# Autodesk Inventor assembly: ma2010_asm
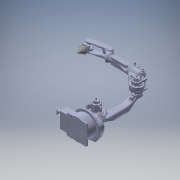
[picture p0: Inventor's stored thumbnail of the model, 180x180]
Saved by Autodesk Inventor 2017 (Build 210142000, 142)
## iProperties
Created: 2020-12-29
Part Number: ma2010_asm
Material: 一般
Document SubType Name: Assembly
Designer: Brian
Sending System: Autodesk Inventor 2020
Preprocessor: ST-DEVELOPER v18
Title: F:\DesktopSpace\MASTERS\ma2010_asm.stp
Author: Crowm
Revision Number: ANY
## Documents named in this file (9)
- E:\Brian\暫存\新增資料夾 (3)\ma2010_asm.iam
- E:\Brian\暫存\新增資料夾 (3)\BASE_AXIS.ipt
- E:\Brian\暫存\新增資料夾 (3)\S_AXIS.ipt
- E:\Brian\暫存\新增資料夾 (3)\L_AXIS.ipt
- E:\Brian\暫存\新增資料夾 (3)\U_AXIS.ipt
- E:\Brian\暫存\新增資料夾 (3)\R_AXIS.ipt
- E:\Brian\暫存\新增資料夾 (3)\B_AXIS.ipt
- E:\Brian\暫存\新增資料夾 (3)\T_AXIS.ipt
- E:\Brian\001\探針.ipt
## Components (8 placed, 8 different names)
1. BASE_AXIS_433 — 貼合:1, 貼合:2, 角度:5
2. S_AXIS_434 — 貼合:1, 貼合:2, 貼合:3, 貼合:4, 角度:2, 角度:3, 角度:4
3. L_AXIS_435 — 貼合:3, 貼合:4, 貼合:5, 貼合:6, 角度:4
4. U_AXIS_436 — 貼合:5, 貼合:6, 貼合:7, 貼合:8, 角度:3
5. R_AXIS_437 — 貼合:7, 貼合:8, 貼合:9, 貼合:10, 角度:1, 角度:2, 角度:5
6. B_AXIS_438 — 貼合:9, 貼合:10, 貼合:11, 貼合:12, 貼合:13, 角度:1
7. T_AXIS_439 — 貼合:11, 貼合:12
8. 探針:1 — 貼合:13
## Relationships (18: Mate 13, Angle 5)
- 貼合:1 [Mate]: BASE_AXIS_433 ↔ S_AXIS_434
- 貼合:2 [Mate]: BASE_AXIS_433 ↔ S_AXIS_434
- 貼合:3 [Mate]: S_AXIS_434 ↔ L_AXIS_435
- 貼合:4 [Mate]: S_AXIS_434 ↔ L_AXIS_435
- 貼合:5 [Mate]: L_AXIS_435 ↔ U_AXIS_436
- 貼合:6 [Mate]: L_AXIS_435 ↔ U_AXIS_436
- 貼合:7 [Mate]: U_AXIS_436 ↔ R_AXIS_437
- 貼合:8 [Mate]: U_AXIS_436 ↔ R_AXIS_437
- 貼合:9 [Mate]: R_AXIS_437 ↔ B_AXIS_438
- 貼合:10 [Mate]: R_AXIS_437 ↔ B_AXIS_438
- 貼合:11 [Mate]: B_AXIS_438 ↔ T_AXIS_439
- 貼合:12 [Mate]: B_AXIS_438 ↔ T_AXIS_439
- 貼合:13 [Mate]: B_AXIS_438 ↔ 探針:1
- 角度:1 [Angle] (180 deg): R_AXIS_437 ↔ B_AXIS_438
- 角度:2 [Angle] (0 deg): S_AXIS_434 ↔ R_AXIS_437
- 角度:3 [Angle] (0 deg): S_AXIS_434 ↔ U_AXIS_436
- 角度:4 [Angle] (0 deg): S_AXIS_434 ↔ L_AXIS_435
- 角度:5 [Angle] (0 deg): BASE_AXIS_433 ↔ R_AXIS_437
